# Autodesk Inventor assembly: Сборка1
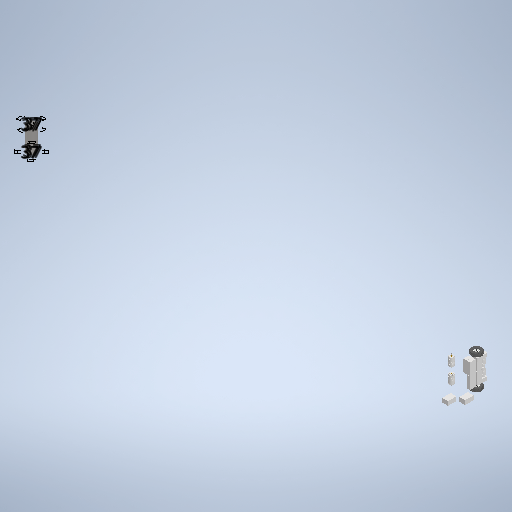
[picture p0: Inventor's stored thumbnail of the model, 512x512]
Saved by Autodesk Inventor 2025.1 (Build 291241000, 241)
## iProperties
Created: 2025-04-09
Part Number: Сборка1
Document SubType Name: Assembly
Designer: tishk
Author: tishk
## Documents named in this file (8)
- C:\Users\tishk\Desktop\Projects\Битва роботов\BOBR\BOBR\Сборка1.iam
- C:\Users\tishk\Desktop\Projects\Битва роботов\BOBR\BOBR\Hobbywing EZrun max4.ipt
- C:\Users\tishk\Desktop\Projects\Битва роботов\BOBR\BOBR\Контроллер EZrun max4.ipt
- C:\Users\tishk\Desktop\Projects\Битва роботов\BOBR\BOBR\Lipo Battery 9500mAh 29.6V.ipt
- C:\Users\tishk\Desktop\Projects\Битва роботов\BOBR\BOBR\Спиннер.ipt
- C:\Users\tishk\Desktop\Projects\Битва роботов\BOBR\BOBR\Крепление Барабана.ipt
- C:\Users\tishk\Desktop\Projects\Битва роботов\BOBR\BOBR\РедукторСмещенный.ipt
- C:\Users\tishk\Desktop\Projects\Битва роботов\BOBR\BOBR\Колесо15.ipt
## Components (18 placed, 7 different names)
1. Hobbywing EZrun max4:1 — Совмещение:25, Совмещение:72, Совмещение:73, Совмещение:76
2. Hobbywing EZrun max4:2 — Совмещение:25, Совмещение:69, Совмещение:70, Совмещение:76
3. Контроллер EZrun max4:1 — Заподлицо:19, Заподлицо:20, Совмещение:75
4. Lipo Battery 9500mAh 29.6V:1 — Заподлицо:24, Заподлицо:25, Заподлицо:27
5. Lipo Battery 9500mAh 29.6V:2 — Совмещение:7, Заподлицо:1, Заподлицо:2, Заподлицо:23, Заподлицо:25, Заподлицо:26, Заподлицо:27
6. Lipo Battery 9500mAh 29.6V:3 — Совмещение:7, Заподлицо:1, Заподлицо:2
7. Hobbywing EZrun max4:3 — Заподлицо:21
8. Hobbywing EZrun max4:4 — Заподлицо:22
9. Контроллер EZrun max4:3
10. Контроллер EZrun max4:4
11. Спиннер:1 — Совмещение:62, Совмещение:63, Совмещение:64, Совмещение:65, Совмещение:66, Совмещение:67, Заподлицо:21, Заподлицо:22
12. Крепление Барабана:1 — Совмещение:62, Совмещение:63, Совмещение:64
13. Крепление Барабана:2 — Совмещение:65, Совмещение:66, Совмещение:67
14. Контроллер EZrun max4:5 — Заподлицо:17, Заподлицо:18, Совмещение:74, Заподлицо:26
15. РедукторСмещенный:1 — Совмещение:68, Заподлицо:15, Совмещение:69, Совмещение:70, Заподлицо:17, Заподлицо:18, Совмещение:74, Заподлицо:23
16. Колесо15:1 — Совмещение:68, Заподлицо:15
17. Колесо15:2 — Совмещение:71, Заподлицо:16
18. РедукторСмещенный:2 — Совмещение:71, Заподлицо:16, Совмещение:72, Совмещение:73, Заподлицо:19, Заподлицо:20, Совмещение:75, Заподлицо:24
## Relationships (33: Mate 18, Flush 15)
- Совмещение:7 [Mate]: Lipo Battery 9500mAh 29.6V:2 ↔ Lipo Battery 9500mAh 29.6V:3
- Заподлицо:1 [Flush]: Lipo Battery 9500mAh 29.6V:2 ↔ Lipo Battery 9500mAh 29.6V:3
- Заподлицо:2 [Flush]: Lipo Battery 9500mAh 29.6V:2 ↔ Lipo Battery 9500mAh 29.6V:3
- Совмещение:25 [Mate]: Hobbywing EZrun max4:1 ↔ Hobbywing EZrun max4:2
- [Mate]: Hobbywing EZrun max4:3 ↔ Hobbywing EZrun max4:4
- Совмещение:62 [Mate]: Спиннер:1 ↔ Крепление Барабана:1
- Совмещение:63 [Mate]: Спиннер:1 ↔ Крепление Барабана:1
- Совмещение:64 [Mate]: Спиннер:1 ↔ Крепление Барабана:1
- Совмещение:65 [Mate]: Спиннер:1 ↔ Крепление Барабана:2
- Совмещение:66 [Mate]: Спиннер:1 ↔ Крепление Барабана:2
- Совмещение:67 [Mate]: Спиннер:1 ↔ Крепление Барабана:2
- Совмещение:68 [Mate]: РедукторСмещенный:1 ↔ Колесо15:1
- Заподлицо:15 [Flush]: РедукторСмещенный:1 ↔ Колесо15:1
- Совмещение:69 [Mate]: Hobbywing EZrun max4:2 ↔ РедукторСмещенный:1
- Совмещение:70 [Mate]: Hobbywing EZrun max4:2 ↔ РедукторСмещенный:1
- Совмещение:71 [Mate]: Колесо15:2 ↔ РедукторСмещенный:2
- Заподлицо:16 [Flush]: Колесо15:2 ↔ РедукторСмещенный:2
- Совмещение:72 [Mate]: Hobbywing EZrun max4:1 ↔ РедукторСмещенный:2
- Совмещение:73 [Mate]: Hobbywing EZrun max4:1 ↔ РедукторСмещенный:2
- Заподлицо:17 [Flush]: Контроллер EZrun max4:5 ↔ РедукторСмещенный:1
- Заподлицо:18 [Flush]: Контроллер EZrun max4:5 ↔ РедукторСмещенный:1
- Совмещение:74 [Mate]: Контроллер EZrun max4:5 ↔ РедукторСмещенный:1
- Заподлицо:19 [Flush]: Контроллер EZrun max4:1 ↔ РедукторСмещенный:2
- Заподлицо:20 [Flush]: Контроллер EZrun max4:1 ↔ РедукторСмещенный:2
- Совмещение:75 [Mate]: Контроллер EZrun max4:1 ↔ РедукторСмещенный:2
- Совмещение:76 [Mate]: Hobbywing EZrun max4:1 ↔ Hobbywing EZrun max4:2
- Заподлицо:21 [Flush]: Hobbywing EZrun max4:3 ↔ Спиннер:1
- Заподлицо:22 [Flush]: Hobbywing EZrun max4:4 ↔ Спиннер:1
- Заподлицо:23 [Flush]: Lipo Battery 9500mAh 29.6V:2 ↔ РедукторСмещенный:1
- Заподлицо:24 [Flush]: Lipo Battery 9500mAh 29.6V:1 ↔ РедукторСмещенный:2
- Заподлицо:25 [Flush]: Lipo Battery 9500mAh 29.6V:1 ↔ Lipo Battery 9500mAh 29.6V:2
- Заподлицо:26 [Flush]: Lipo Battery 9500mAh 29.6V:2 ↔ Контроллер EZrun max4:5
- Заподлицо:27 [Flush]: Lipo Battery 9500mAh 29.6V:1 ↔ Lipo Battery 9500mAh 29.6V:2
## Named parameters: d73_d26 = 0 mm
